# Autodesk Inventor assembly: 100-10-FRAME-TOP-01
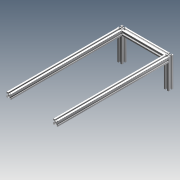
[picture p0: Inventor's stored thumbnail of the model, 180x180]
Saved by Autodesk Inventor 2018.2 (Build 222227000, 227)
## iProperties
Manager: feesmrt
Company: FRANCOR
Part Number: 100-10-FRAME-TOP-01
Project: Rescue Robot
Cost Center: -
Material: Generisch
Document SubType Name: Assembly
Designer: feesmrt
Engineer: feesmrt
Authority: feesmrt
Subject: Rescue Robot
Author: feesmrt
Revision Number: 1
## Documents named in this file (4)
- D:\Programmierung\FRANC0R\CAD\02-Rocker-Bogie-Robot\100-CHASSIS\10-FRAME\100-10-FRAME-TOP-01.iam
- D:\Programmierung\FRANC0R\CAD\02-Rocker-Bogie-Robot\100-CHASSIS\10-FRAME\100-10-FRAME-PROFILE-TOP-W-01.ipt
- D:\Programmierung\FRANC0R\CAD\02-Rocker-Bogie-Robot\100-CHASSIS\10-FRAME\100-10-FRAME-PROFILE-TOP-H-01.ipt
- D:\Programmierung\FRANC0R\CAD\02-Rocker-Bogie-Robot\100-CHASSIS\10-FRAME\100-10-FRAME-PROFILE-TOP-L-01.ipt
## Components (5 placed, 3 different names)
1. 100-10-FRAME-PROFILE-TOP-W-01:1 — Passend:1, Passend:2, Fluchtend:1, Fluchtend:2, Fluchtend:3, Fluchtend:4
2. 100-10-FRAME-PROFILE-TOP-H-01:1 — Passend:1, Fluchtend:3, Fluchtend:4, Passend:4, Fluchtend:5, Fluchtend:6
3. 100-10-FRAME-PROFILE-TOP-H-01:2 — Passend:2, Fluchtend:1, Fluchtend:2, Passend:3, Fluchtend:7, Fluchtend:8
4. 100-10-FRAME-PROFILE-TOP-L-01:1 — Passend:4, Fluchtend:5, Fluchtend:6
5. 100-10-FRAME-PROFILE-TOP-L-01:2 — Passend:3, Fluchtend:7, Fluchtend:8
## Relationships (12: Flush 8, Mate 4)
- Passend:1 [Mate]: 100-10-FRAME-PROFILE-TOP-W-01:1 ↔ 100-10-FRAME-PROFILE-TOP-H-01:1
- Passend:2 [Mate]: 100-10-FRAME-PROFILE-TOP-W-01:1 ↔ 100-10-FRAME-PROFILE-TOP-H-01:2
- Fluchtend:1 [Flush]: 100-10-FRAME-PROFILE-TOP-W-01:1 ↔ 100-10-FRAME-PROFILE-TOP-H-01:2
- Fluchtend:2 [Flush]: 100-10-FRAME-PROFILE-TOP-W-01:1 ↔ 100-10-FRAME-PROFILE-TOP-H-01:2
- Fluchtend:3 [Flush]: 100-10-FRAME-PROFILE-TOP-W-01:1 ↔ 100-10-FRAME-PROFILE-TOP-H-01:1
- Fluchtend:4 [Flush]: 100-10-FRAME-PROFILE-TOP-W-01:1 ↔ 100-10-FRAME-PROFILE-TOP-H-01:1
- Passend:3 [Mate]: 100-10-FRAME-PROFILE-TOP-H-01:2 ↔ 100-10-FRAME-PROFILE-TOP-L-01:2
- Passend:4 [Mate]: 100-10-FRAME-PROFILE-TOP-H-01:1 ↔ 100-10-FRAME-PROFILE-TOP-L-01:1
- Fluchtend:5 [Flush]: 100-10-FRAME-PROFILE-TOP-H-01:1 ↔ 100-10-FRAME-PROFILE-TOP-L-01:1
- Fluchtend:6 [Flush]: 100-10-FRAME-PROFILE-TOP-H-01:1 ↔ 100-10-FRAME-PROFILE-TOP-L-01:1
- Fluchtend:7 [Flush]: 100-10-FRAME-PROFILE-TOP-H-01:2 ↔ 100-10-FRAME-PROFILE-TOP-L-01:2
- Fluchtend:8 [Flush]: 100-10-FRAME-PROFILE-TOP-H-01:2 ↔ 100-10-FRAME-PROFILE-TOP-L-01:2
